# Autodesk Inventor assembly: Turret ASM
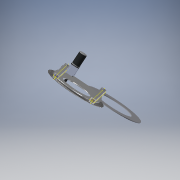
[picture p0: Inventor's stored thumbnail of the model, 180x180]
Saved by Autodesk Inventor 2017 (Build 210142000, 142)
## iProperties
Created: 2016-09-26
Part Number: Turret ASM
Document SubType Name: Assembly
Designer: Hanson
Author: Hanson
## Documents named in this file (14)
- \\Mac\Home\Desktop\bunnybots 2016\15102898-16-Bunnybot-CAD\Bunnybot-To_be_renamed\15102898-16-A-0000\15102898-16-A-0600\Turret ASM.iam
- \\Mac\Home\Desktop\bunnybots 2016\15102898-16-Bunnybot-CAD\Bunnybot-To_be_renamed\15102898-16-A-0000\15102898-16-A-0600\User Library-LazySusan 12inch.ipt
- \\Mac\Home\Desktop\bunnybots 2016\15102898-16-Bunnybot-CAD\Bunnybot-To_be_renamed\15102898-16-A-0000\15102898-16-A-0600\Large crossbeam.ipt
- \\Mac\Home\Desktop\bunnybots 2016\15102898-16-Bunnybot-CAD\Bunnybot-To_be_renamed\15102898-16-A-0000\15102898-16-A-0600\90480A195_LOW-STRENGTH STEEL HEX NUT.ipt
- \\Mac\Home\Desktop\bunnybots 2016\15102898-16-Bunnybot-CAD\Bunnybot-To_be_renamed\15102898-16-A-0000\15102898-16-A-0600\92196A277_18-8 STAINLESS STEEL SOCKET HEAD CAP SCREW.ipt
- \\Mac\Home\Desktop\bunnybots 2016\15102898-16-Bunnybot-CAD\Bunnybot-To_be_renamed\15102898-16-A-0000\15102898-16-A-0600\BAG motor top plate.ipt
- \\Mac\Home\Desktop\bunnybots 2016\15102898-16-Bunnybot-CAD\Bunnybot-To_be_renamed\15102898-16-A-0000\15102898-16-A-0600\92196A545_18-8 STAINLESS STEEL SOCKET HEAD CAP SCREW.ipt
- \\Mac\Home\Desktop\bunnybots 2016\15102898-16-Bunnybot-CAD\Bunnybot-To_be_renamed\15102898-16-A-0000\15102898-16-A-0600\plate mount nut.ipt
- \\Mac\Home\Desktop\bunnybots 2016\15102898-16-Bunnybot-CAD\Bunnybot-To_be_renamed\15102898-16-A-0000\15102898-16-A-0600\lazy susan bushing.ipt
- \\Mac\Home\Desktop\bunnybots 2016\15102898-16-Bunnybot-CAD\Bunnybot-To_be_renamed\15102898-16-A-0000\15102898-16-A-0600\BAG motor\VersaPlanetary-1-Stage-with-BAG-Motor.iam
- \\Mac\Home\Desktop\bunnybots 2016\15102898-16-Bunnybot-CAD\Bunnybot-To_be_renamed\15102898-16-A-0000\15102898-16-A-0600\217-2642-STEP-20140807.ipt
- \\Mac\Home\Desktop\bunnybots 2016\15102898-16-Bunnybot-CAD\Bunnybot-To_be_renamed\15102898-16-A-0000\15102898-16-A-0600\support ring.ipt
- \\Mac\Home\Desktop\bunnybots 2016\15102898-16-Bunnybot-CAD\Bunnybot-To_be_renamed\15102898-16-A-0000\15102898-16-A-0600\roundplate.ipt
- \\Mac\Home\Desktop\bunnybots 2016\15102898-16-Bunnybot-CAD\Bunnybot-To_be_renamed\15102898-16-A-0000\15102898-16-A-0600\Turret ASM\Design Accelerator\Chain Drive3.iam
## Components (18 placed, 13 different names)
1. User Library-LazySusan 12inch:1 — Mate:5, Mate:7, Mate:10, Mate:25, Mate:26, Mate:27, Mate:28, Mate:29
2. Large crossbeam:1 — Insert:16, Flush:1, Flush:2, Mate:17, Flush:3
3. Large crossbeam:2 — Insert:13, Insert:14, Insert:15, Flush:1, Mate:14, Flush:2, Mate:19, Flush:6
4. 92196A277_18-8 STAINLESS STEEL SOCKET HEAD CAP SCREW:1 — Insert:13
5. 92196A277_18-8 STAINLESS STEEL SOCKET HEAD CAP SCREW:2 — Insert:14
6. BAG motor top plate:1 — Insert:11, Insert:12, Mate:14, Flush:3, Mate:18, Flush:4, Flush:6, Mate:25, Mate:26, Mate:27, Mate:30
7. 92196A545_18-8 STAINLESS STEEL SOCKET HEAD CAP SCREW:1 — Insert:11
8. 92196A545_18-8 STAINLESS STEEL SOCKET HEAD CAP SCREW:2 — Insert:12, Mate:17
9. plate mount nut:1 — Insert:15
10. plate mount nut:2 — Insert:16
11. lazy susan bushing:1 — Mate:5, Mate:24
12. 90480A195_LOW-STRENGTH STEEL HEX NUT:2 — Mate:7, Mate:24
13. 90480A195_LOW-STRENGTH STEEL HEX NUT:4 — Mate:10
14. VersaPlanetary-1-Stage-with-BAG-Motor:1 [sub-assembly] — Mate:18, Mate:19, Flush:4, Mate:20, Mate:21
15. 217-2642-STEP-20140807:1 — Mate:20, Mate:21, Flush:7
16. support ring:1 — Mate:28, Mate:29, Mate:30, Mate:31, Mate:32, Mate:33
17. roundplate:1 — Mate:31, Mate:32, Mate:33, Flush:7
18. Chain Drive:1 [sub-assembly]
## Relationships (31: Mate 19, Insert 6, Flush 6)
- Insert:11: BAG motor top plate:1 ↔ 92196A545_18-8 STAINLESS STEEL SOCKET HEAD CAP SCREW:1
- Insert:12: BAG motor top plate:1 ↔ 92196A545_18-8 STAINLESS STEEL SOCKET HEAD CAP SCREW:2
- Insert:13: Large crossbeam:2 ↔ 92196A277_18-8 STAINLESS STEEL SOCKET HEAD CAP SCREW:1
- Insert:14: Large crossbeam:2 ↔ 92196A277_18-8 STAINLESS STEEL SOCKET HEAD CAP SCREW:2
- Insert:15: Large crossbeam:2 ↔ plate mount nut:1
- Insert:16: Large crossbeam:1 ↔ plate mount nut:2
- Flush:1: Large crossbeam:1 ↔ Large crossbeam:2
- Mate:5: User Library-LazySusan 12inch:1 ↔ lazy susan bushing:1
- Mate:7: User Library-LazySusan 12inch:1 ↔ 90480A195_LOW-STRENGTH STEEL HEX NUT:2
- Mate:10: User Library-LazySusan 12inch:1 ↔ 90480A195_LOW-STRENGTH STEEL HEX NUT:4
- Mate:14: Large crossbeam:2 ↔ BAG motor top plate:1
- Flush:2: Large crossbeam:1 ↔ Large crossbeam:2
- Mate:17: Large crossbeam:1 ↔ 92196A545_18-8 STAINLESS STEEL SOCKET HEAD CAP SCREW:2
- Flush:3: Large crossbeam:1 ↔ BAG motor top plate:1
- Mate:18: BAG motor top plate:1 ↔ VersaPlanetary-1-Stage-with-BAG-Motor:1
- Mate:19: Large crossbeam:2 ↔ VersaPlanetary-1-Stage-with-BAG-Motor:1
- Flush:4: BAG motor top plate:1 ↔ VersaPlanetary-1-Stage-with-BAG-Motor:1
- Mate:20: VersaPlanetary-1-Stage-with-BAG-Motor:1 ↔ 217-2642-STEP-20140807:1
- Mate:21: VersaPlanetary-1-Stage-with-BAG-Motor:1 ↔ 217-2642-STEP-20140807:1
- Mate:24: lazy susan bushing:1 ↔ 90480A195_LOW-STRENGTH STEEL HEX NUT:2
- Flush:6: Large crossbeam:2 ↔ BAG motor top plate:1
- Mate:25: User Library-LazySusan 12inch:1 ↔ BAG motor top plate:1
- Mate:26: User Library-LazySusan 12inch:1 ↔ BAG motor top plate:1
- Mate:27: User Library-LazySusan 12inch:1 ↔ BAG motor top plate:1
- Mate:28: User Library-LazySusan 12inch:1 ↔ support ring:1
- Mate:29: User Library-LazySusan 12inch:1 ↔ support ring:1
- Mate:30: BAG motor top plate:1 ↔ support ring:1
- Mate:31: support ring:1 ↔ roundplate:1
- Mate:32: support ring:1 ↔ roundplate:1
- Mate:33: support ring:1 ↔ roundplate:1
- Flush:7: 217-2642-STEP-20140807:1 ↔ roundplate:1
